# Autodesk Inventor assembly: Free Sprocket Holder
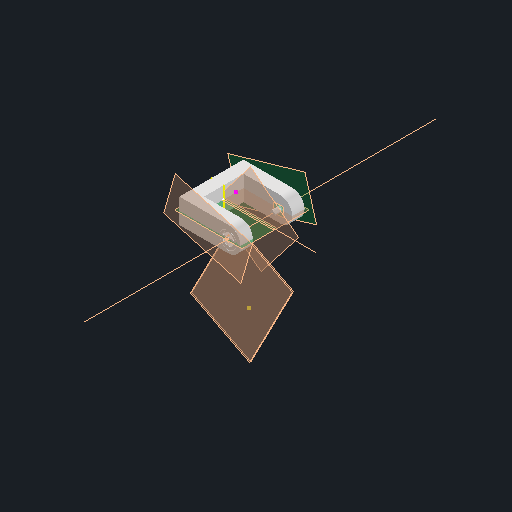
[picture p0: Inventor's stored thumbnail of the model, 512x512]
Saved by Autodesk Inventor 2025.2 (Build 292293000, 293)
## iProperties
Created: 2024-11-16
Part Number: Free Sprocket Holder
Document SubType Name: Assembly
Designer: JL
Author: JL
## Documents named in this file (3)
- C:\Users\ModEn\Documents\University\Aalto\DTEP\Inventor Projects\Curtain Opener - Copy\Free Sprocket Holder.iam
- C:\Users\ModEn\Documents\University\Aalto\DTEP\Inventor Projects\Curtain Opener - Copy\Free Sprocket Holder Body.ipt
- C:\Users\ModEn\Documents\University\Aalto\DTEP\Inventor Projects\Curtain Opener - Copy\Axle Screw.ipt
## Components (3 placed, 2 different names)
1. Free Sprocket Holder Body:1 — Mate:1, Mate:2, Flush:1, Flush:2, Mate:3, Mate:4, Mate:5
2. Axle Screw:1 — Flush:1, Flush:2
3. Axle Screw:2 — Mate:3, Mate:4, Mate:5
## Relationships (7: Mate 5, Flush 2)
- Mate:1: Free Sprocket Holder Body:1
- Mate:2: Free Sprocket Holder Body:1
- Flush:1: Free Sprocket Holder Body:1 ↔ Axle Screw:1
- Flush:2: Free Sprocket Holder Body:1 ↔ Axle Screw:1
- Mate:3: Free Sprocket Holder Body:1 ↔ Axle Screw:2
- Mate:4: Free Sprocket Holder Body:1 ↔ Axle Screw:2
- Mate:5: Free Sprocket Holder Body:1 ↔ Axle Screw:2
